# Autodesk Inventor assembly: SmallContainerAssembly
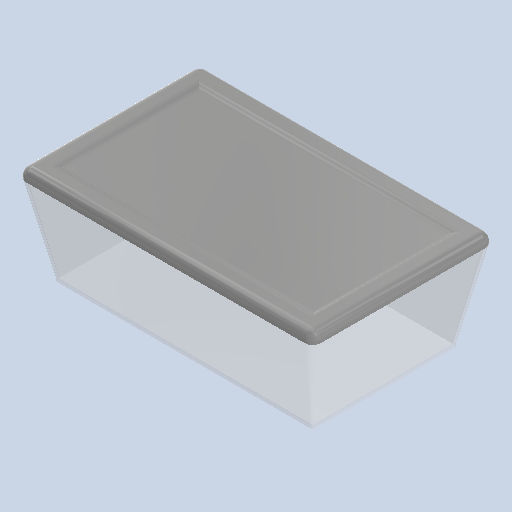
[picture p0: Inventor's stored thumbnail of the model, 512x512]
Saved by Autodesk Inventor 2024 (Build 280153000, 153)
## iProperties
Created: 2023-06-09
Part Number: SmallContainerAssembly
Document SubType Name: Assembly
Designer: 18179
Author: 18179
## Documents named in this file (3)
- C:\Users\18179\Desktop\TuppyMkIV\SmallContainerAssembly.iam
- C:\Users\18179\Desktop\TuppyMkIV\SmallContainer.ipt
- C:\Users\18179\Desktop\TuppyMkIV\SmallContainerLid.ipt
## Components (2 placed, 2 different names)
1. SmallContainer:1 — Mate:1, Mate:2, Mate:3
2. SmallContainerLid:1 — Mate:1, Mate:2, Mate:3
## Relationships (3: Mate 3)
- Mate:1: SmallContainer:1 ↔ SmallContainerLid:1
- Mate:2: SmallContainer:1 ↔ SmallContainerLid:1
- Mate:3: SmallContainer:1 ↔ SmallContainerLid:1
